# Autodesk Inventor assembly: support
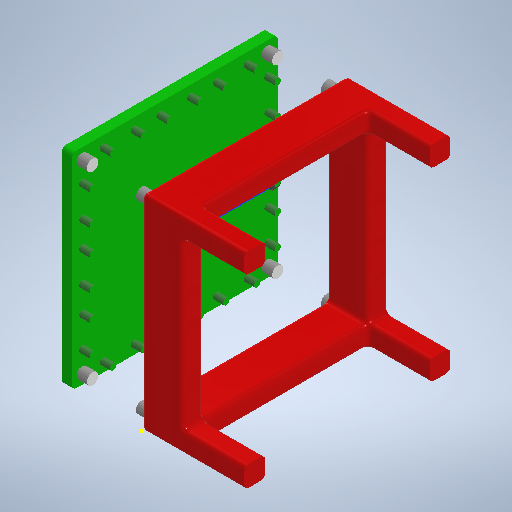
[picture p0: Inventor's stored thumbnail of the model, 512x512]
Saved by Autodesk Inventor 2025 (Build 290162010, 162A)
## iProperties
Created: 2025-02-15
Part Number: support
Document SubType Name: Assembly
Designer: antoi
Author: antoi
## Documents named in this file (6)
- C:\projet table\clone\support.iam
- C:\projet table\clone\Pièce1.ipt
- C:\projet table\clone\vis.ipt
- C:\projet table\clone\plateau.ipt
- C:\projet table\clone\DFR0440.ipt
- C:\Users\arthu\Documents\Inventor\Content Center Files\R2025\fr-FR\ISO 4036(2)\ISO 4036 - M3.5 _(2).ipt
## Components (13 placed, 5 different names)
1. Pièce1:1 — Affleurement:1, Placage:1, Placage:2, Placage:3, Placage:4, Affleurement:2, Affleurement:3, Affleurement:4, Affleurement:5
2. vis:1 — Placage:3, Affleurement:2, Placage:5
3. vis:2 — Placage:4, Affleurement:3
4. vis:3 — Placage:2, Affleurement:5, Placage:6
5. vis:4 — Placage:1, Affleurement:4
6. plateau:1 — Placage:5, Placage:6, Placage:7, Placage:8, Cylindrique:1, Cylindrique:3, Cylindrique:4, Cylindrique:5, Affleurement:6, Affleurement:7, Affleurement:8, Affleurement:9, Placage:9, Placage:10, Placage:12
7. DFR0440:1 — Placage:7, Placage:8, Placage:9, Placage:11, Placage:13
8. vis:5 — Cylindrique:3, Affleurement:8
9. vis:6 — Cylindrique:5, Affleurement:7
10. vis:7 — Cylindrique:4, Affleurement:9
11. vis:8 — Cylindrique:1, Affleurement:6
12. ISO 4036 M3.5 *:1 — Placage:10, Placage:11
13. ISO 4036 M3.5 *:2 — Placage:12, Placage:13
## Relationships (26: Mate 13, Flush 9, CylindricalJoint 4)
- Affleurement:1 [Flush] (-5 mm): Pièce1:1
- Placage:1 [Mate]: Pièce1:1 ↔ vis:4
- Placage:2 [Mate]: Pièce1:1 ↔ vis:3
- Placage:3 [Mate]: Pièce1:1 ↔ vis:1
- Placage:4 [Mate]: Pièce1:1 ↔ vis:2
- Affleurement:2 [Flush] (-5 mm): Pièce1:1 ↔ vis:1
- Affleurement:3 [Flush] (-5 mm): Pièce1:1 ↔ vis:2
- Affleurement:4 [Flush] (5 mm): Pièce1:1 ↔ vis:4
- Affleurement:5 [Flush] (-5 mm): Pièce1:1 ↔ vis:3
- Placage:5 [Mate]: vis:1 ↔ plateau:1
- Placage:6 [Mate]: vis:3 ↔ plateau:1
- Placage:7 [Mate]: plateau:1 ↔ DFR0440:1
- Placage:8 [Mate]: plateau:1 ↔ DFR0440:1
- Cylindrique:1: plateau:1 ↔ vis:8
- Cylindrique:3: plateau:1 ↔ vis:5
- Cylindrique:4: plateau:1 ↔ vis:7
- Cylindrique:5: plateau:1 ↔ vis:6
- Affleurement:6 [Flush]: plateau:1 ↔ vis:8
- Affleurement:7 [Flush]: plateau:1 ↔ vis:6
- Affleurement:8 [Flush]: plateau:1 ↔ vis:5
- Affleurement:9 [Flush]: plateau:1 ↔ vis:7
- Placage:9 [Mate]: plateau:1 ↔ DFR0440:1
- Placage:10 [Mate]: plateau:1 ↔ ISO 4036 M3.5 *:1
- Placage:11 [Mate]: DFR0440:1 ↔ ISO 4036 M3.5 *:1
- Placage:12 [Mate]: plateau:1 ↔ ISO 4036 M3.5 *:2
- Placage:13 [Mate]: DFR0440:1 ↔ ISO 4036 M3.5 *:2
